# Autodesk Inventor assembly: 22nc_kadotome_4
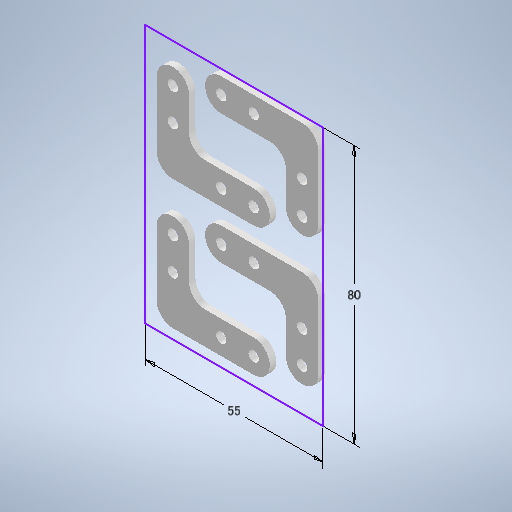
[picture p0: Inventor's stored thumbnail of the model, 512x512]
Saved by Autodesk Inventor 2025.1 (Build 291241000, 241)
## iProperties
Created: 2025-05-06
Part Number: 22nc_kadotome_4
Document SubType Name: Assembly
Designer: yuki0520
Author: yuki0520
## Documents named in this file (2)
- C:\Users\yuki0520\OneDrive\ドキュメント\Inventor\2025_nhk\tanaka\nageru\light\22nc_kadotome_4.iam
- C:\Users\yuki0520\OneDrive\ドキュメント\Inventor\2025_nhk\tanaka\nageru\smallring\kakutome_nc.ipt
## Components (4 placed, 1 different names)
1. kakutome_nc:1 — フラッシュ:1, フラッシュ:2, フラッシュ:3, メイト:1, メイト:2, フラッシュ:4
2. kakutome_nc:2 — フラッシュ:1, メイト:1, メイト:2, メイト:5
3. kakutome_nc:3 — フラッシュ:2, メイト:3, メイト:4, フラッシュ:4, メイト:5
4. kakutome_nc:4 — フラッシュ:3, メイト:3, メイト:4
## Relationships (9: Mate 5, Flush 4)
- フラッシュ:1 [Flush]: kakutome_nc:1 ↔ kakutome_nc:2
- フラッシュ:2 [Flush]: kakutome_nc:1 ↔ kakutome_nc:3
- フラッシュ:3 [Flush]: kakutome_nc:1 ↔ kakutome_nc:4
- メイト:1 [Mate] (15 mm): kakutome_nc:1 ↔ kakutome_nc:2
- メイト:2 [Mate] (30 mm): kakutome_nc:1 ↔ kakutome_nc:2
- メイト:3 [Mate] (15 mm): kakutome_nc:3 ↔ kakutome_nc:4
- メイト:4 [Mate] (30 mm): kakutome_nc:3 ↔ kakutome_nc:4
- フラッシュ:4 [Flush]: kakutome_nc:1 ↔ kakutome_nc:3
- メイト:5 [Mate] (5 mm): kakutome_nc:2 ↔ kakutome_nc:3
